# Autodesk Inventor assembly: POM_T5_07
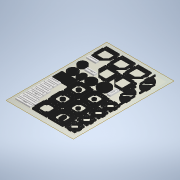
[picture p0: Inventor's stored thumbnail of the model, 180x180]
Saved by Autodesk Inventor 2020 (Build 240168000, 168)
## iProperties
Created: 2021-08-27
Part Number: POM_T5_07
Document SubType Name: Assembly
Designer: Masato
Author: Masato
## Documents named in this file (26)
- C:\Inventor\SUSTAINA-OP\Cam\POM_T5_07.iam
- C:\Inventor\SUSTAINA-OP\Cam\DisposableBoard.ipt
- C:\Inventor\SUSTAINA-OP\UpperBody\Head\Camera_root_frame_e-CAM50_CUNX.ipt
- C:\Inventor\SUSTAINA-OP\UpperBody\Arm\UpperArm_diagonal.ipt
- C:\Inventor\SUSTAINA-OP\UpperBody\Head\Camera_side_frame.ipt
- C:\Inventor\SUSTAINA-OP\SandBlastingJig\Trunk_servo_bottom_frame_SandBlastingJig.ipt
- C:\Inventor\SUSTAINA-OP\SandBlastingJig\Foot_front_frame_SandBlastingJig_back.ipt
- C:\Inventor\SUSTAINA-OP\SandBlastingJig\Foot_front_frame_SandBlastingJig_front.ipt
- C:\Inventor\SUSTAINA-OP\SandBlastingJig\Leg_joint_slider_frame_SandBlastingJig_axis_back.ipt
- C:\Inventor\SUSTAINA-OP\SandBlastingJig\Leg_joint_slider_frame_SandBlastingJig_axis_front.ipt
- C:\Inventor\SUSTAINA-OP\SandBlastingJig\Leg_joint_slider_frame_SandBlastingJig_slider_back.ipt
- C:\Inventor\SUSTAINA-OP\SandBlastingJig\Leg_joint_slider_frame_SandBlastingJig_slider_front.ipt
- C:\Inventor\SUSTAINA-OP\SandBlastingJig\Leg_joint_yaw_frame_SandBlastingJig.ipt
- C:\Inventor\SUSTAINA-OP\SandBlastingJig\Outer_support_stand_SandBlastingJig.ipt
- C:\Inventor\SUSTAINA-OP\SandBlastingJig\Shoulder_horn_frame_SandBlastingJig.ipt
- C:\Inventor\SUSTAINA-OP\SandBlastingJig\Trunk_neck_frame_AND_Trunk_shoulder_frame_SandBlastingJig.ipt
- C:\Inventor\SUSTAINA-OP\UpperBody\Arm\ForeArm_diagonal.ipt
- C:\Inventor\SUSTAINA-OP\Jig\BackLink_diagonal_Jig.ipt
- C:\Inventor\SUSTAINA-OP\Jig\Leg_joint_yaw_frame_Jig.ipt
- C:\Inventor\SUSTAINA-OP\Jig\Trunk_lower_side_frame_Jig.ipt
- C:\Inventor\SUSTAINA-OP\Jig\FrontLink_diagonal_Jig.ipt
- C:\Inventor\SUSTAINA-OP\Jig\Trunk_chest_frame_Jig_1.ipt
- C:\Inventor\SUSTAINA-OP\Jig\UpperArm_diagonal_Jig.ipt
- C:\Inventor\SUSTAINA-OP\Jig\Head_horn_frame_Jig.ipt
- C:\Inventor\SUSTAINA-OP\Jig\Shoulder_horn_frame_Jig.ipt
- C:\Inventor\SUSTAINA-OP\Jig\Foot_root_block_Jig.ipt
## Components (43 placed, 25 different names)
1. DisposableBoard:1 — メイト:2, メイト:1, フラッシュ:1, フラッシュ:2, メイト:4, メイト:5, メイト:6, メイト:7, メイト:8, メイト:9, メイト:13, メイト:14, メイト:16, メイト:17, メイト:20, メイト:22, メイト:23, メイト:25, メイト:26, メイト:27, メイト:28, 角度:1, 角度:2, 角度:3, 角度:4, メイト:29, 角度:5, メイト:30, メイト:31, メイト:32, メイト:33, メイト:34, メイト:35, フラッシュ:3, フラッシュ:4, 角度:6, 角度:7, 角度:8, 角度:9, 角度:10, 正接:11, 正接:19, メイト:36, フラッシュ:5, フラッシュ:6, メイト:38, メイト:41, フラッシュ:7, メイト:49, 角度:11, メイト:52, メイト:54, フラッシュ:9, フラッシュ:10, メイト:55, メイト:57, メイト:59, メイト:61, メイト:63, メイト:65, メイト:67, メイト:69
2. Camera_side_frame:1 — メイト:13, メイト:14, メイト:15, メイト:19
3. Camera_side_frame:4 — メイト:17, メイト:20, メイト:24, メイト:50
4. Camera_side_frame:5 — メイト:16, メイト:19, メイト:40, メイト:50, フラッシュ:8
5. Camera_side_frame:6 — メイト:22, メイト:23, メイト:24, フラッシュ:8
6. Trunk_servo_bottom_frame_SandBlastingJig:1 — メイト:30, フラッシュ:3, フラッシュ:4, 正接:12, 正接:13
7. Foot_front_frame_SandBlastingJig_back:1 — メイト:26, 角度:3, 正接:5, 正接:6
8. Foot_front_frame_SandBlastingJig_front:1 — メイト:25, 角度:2, 正接:1, 正接:2
9. Leg_joint_slider_frame_SandBlastingJig_axis_back:1 — メイト:27, 角度:4, 正接:7, 正接:8
10. Leg_joint_slider_frame_SandBlastingJig_axis_front:1 — メイト:28, 角度:1, 正接:3, 正接:4
11. Leg_joint_slider_frame_SandBlastingJig_slider_back:1 — メイト:29, 角度:5, 正接:9, 正接:10
12. Leg_joint_slider_frame_SandBlastingJig_slider_front:1 — メイト:32, 角度:7, 正接:13, 正接:14, 正接:15
13. Leg_joint_yaw_frame_SandBlastingJig:1 — メイト:33, 角度:10, 正接:19, 正接:20, 正接:21
14. Outer_support_stand_SandBlastingJig:1 — メイト:35, 角度:9, 正接:17, 正接:18, 正接:22
15. Shoulder_horn_frame_SandBlastingJig:1 — メイト:34, 角度:8, 正接:15, 正接:16, 正接:17
16. Trunk_neck_frame_AND_Trunk_shoulder_frame_SandBlastingJig:1 — メイト:31, 角度:6, 正接:11, 正接:12, 正接:14, 正接:20
17. BackLink_diagonal_Jig:1 — メイト:41, フラッシュ:7, メイト:46
18. Leg_joint_yaw_frame_Jig:1 — メイト:49, メイト:51, 角度:11, 正接:21
19. Leg_joint_yaw_frame_Jig:2 — メイト:52, メイト:53, 正接:22
20. Trunk_lower_side_frame_Jig:1 — メイト:54, フラッシュ:9, フラッシュ:10, メイト:56, フラッシュ:11
21. FrontLink_diagonal_Jig:1 — メイト:55, メイト:56, フラッシュ:11, メイト:58, フラッシュ:12
22. Trunk_chest_frame_Jig_1:1 — メイト:57, メイト:58, フラッシュ:12, メイト:60, フラッシュ:13
23. UpperArm_diagonal_Jig:1 — メイト:59, メイト:60, フラッシュ:13, メイト:62, フラッシュ:14
24. Head_horn_frame_Jig:1 — メイト:61, メイト:62, フラッシュ:14, メイト:64, フラッシュ:15
25. Shoulder_horn_frame_Jig:1 — メイト:63, メイト:64, フラッシュ:15, メイト:66, フラッシュ:16
26. BackLink_diagonal_Jig:2 — メイト:65, メイト:66, フラッシュ:16, メイト:68, フラッシュ:17
27. Leg_joint_yaw_frame_Jig:3 — メイト:67, メイト:68, フラッシュ:17, メイト:70, フラッシュ:18
28. Foot_root_block_Jig:1 — メイト:69, メイト:70, フラッシュ:18
29. UpperArm_diagonal:1 — メイト:7, メイト:8, メイト:9
30. UpperArm_diagonal:2
31. UpperArm_diagonal:3
32. UpperArm_diagonal:4 — メイト:15
33. ForeArm_diagonal:1 — メイト:36, フラッシュ:5, フラッシュ:6, メイト:46
34. ForeArm_diagonal:2
35. ForeArm_diagonal:3 — メイト:39
36. ForeArm_diagonal:4 — メイト:38, メイト:39, メイト:40, メイト:53
37. ForeArm_diagonal:5 — メイト:51
38. Camera_root_frame_e-CAM50_CUNX:1 — メイト:4, メイト:5, メイト:6
39. Camera_root_frame_e-CAM50_CUNX:2 — 正接:9, 正接:10
40. Camera_root_frame_e-CAM50_CUNX:3 — 正接:1, 正接:2
41. Camera_root_frame_e-CAM50_CUNX:4 — 正接:3, 正接:4
42. Camera_root_frame_e-CAM50_CUNX:5 — 正接:5, 正接:6, 正接:16
43. Camera_root_frame_e-CAM50_CUNX:6 — 正接:7, 正接:8, 正接:18
## Component patterns: (4 elements, first: UpperArm_diagonal:1), (3 elements), (3 elements, first: ForeArm_diagonal:1), (2 elements, first: ForeArm_diagonal:4), (2 elements, first: Camera_root_frame_e-CAM50_CUNX:1), コンポーネント パターン 7:2 (2 elements), コンポーネント パターン 7:3 (2 elements)
## Relationships (108: Mate 57, Tangent 22, Flush 18, Angle 11)
- メイト:2 [Mate]: DisposableBoard:1
- メイト:1 [Mate]: DisposableBoard:1
- フラッシュ:1 [Flush]: DisposableBoard:1
- フラッシュ:2 [Flush]: DisposableBoard:1
- メイト:4 [Mate]: DisposableBoard:1 ↔ Camera_root_frame_e-CAM50_CUNX:1
- メイト:5 [Mate] (2 mm): DisposableBoard:1 ↔ Camera_root_frame_e-CAM50_CUNX:1
- メイト:6 [Mate] (56.2 mm): DisposableBoard:1 ↔ Camera_root_frame_e-CAM50_CUNX:1
- メイト:7 [Mate]: DisposableBoard:1 ↔ UpperArm_diagonal:1
- メイト:8 [Mate] (2 mm): DisposableBoard:1 ↔ UpperArm_diagonal:1
- メイト:9 [Mate] (2 mm): DisposableBoard:1 ↔ UpperArm_diagonal:1
- メイト:13 [Mate]: DisposableBoard:1 ↔ Camera_side_frame:1
- メイト:14 [Mate] (5 mm): DisposableBoard:1 ↔ Camera_side_frame:1
- メイト:15 [Mate] (2.5 mm): Camera_side_frame:1 ↔ UpperArm_diagonal:4
- メイト:16 [Mate]: DisposableBoard:1 ↔ Camera_side_frame:5
- メイト:17 [Mate]: DisposableBoard:1 ↔ Camera_side_frame:4
- メイト:19 [Mate] (10 mm): Camera_side_frame:1 ↔ Camera_side_frame:5
- メイト:20 [Mate] (5 mm): DisposableBoard:1 ↔ Camera_side_frame:4
- メイト:22 [Mate]: DisposableBoard:1 ↔ Camera_side_frame:6
- メイト:23 [Mate] (2 mm): DisposableBoard:1 ↔ Camera_side_frame:6
- メイト:24 [Mate] (9 mm): Camera_side_frame:4 ↔ Camera_side_frame:6
- メイト:25 [Mate]: DisposableBoard:1 ↔ Foot_front_frame_SandBlastingJig_front:1
- メイト:26 [Mate]: DisposableBoard:1 ↔ Foot_front_frame_SandBlastingJig_back:1
- メイト:27 [Mate]: DisposableBoard:1 ↔ Leg_joint_slider_frame_SandBlastingJig_axis_back:1
- メイト:28 [Mate]: DisposableBoard:1 ↔ Leg_joint_slider_frame_SandBlastingJig_axis_front:1
- 角度:1 [Angle] (0 deg): DisposableBoard:1 ↔ Leg_joint_slider_frame_SandBlastingJig_axis_front:1
- 角度:2 [Angle] (0 deg): DisposableBoard:1 ↔ Foot_front_frame_SandBlastingJig_front:1
- 角度:3 [Angle] (0 deg): DisposableBoard:1 ↔ Foot_front_frame_SandBlastingJig_back:1
- 角度:4 [Angle] (0 deg): DisposableBoard:1 ↔ Leg_joint_slider_frame_SandBlastingJig_axis_back:1
- 正接:1 [Tangent] (7.5 mm): Foot_front_frame_SandBlastingJig_front:1 ↔ Camera_root_frame_e-CAM50_CUNX:3
- 正接:2 [Tangent] (7.5 mm): Foot_front_frame_SandBlastingJig_front:1 ↔ Camera_root_frame_e-CAM50_CUNX:3
- 正接:3 [Tangent] (7.5 mm): Leg_joint_slider_frame_SandBlastingJig_axis_front:1 ↔ Camera_root_frame_e-CAM50_CUNX:4
- 正接:4 [Tangent] (7.5 mm): Leg_joint_slider_frame_SandBlastingJig_axis_front:1 ↔ Camera_root_frame_e-CAM50_CUNX:4
- 正接:5 [Tangent] (7.5 mm): Foot_front_frame_SandBlastingJig_back:1 ↔ Camera_root_frame_e-CAM50_CUNX:5
- 正接:6 [Tangent] (7.5 mm): Foot_front_frame_SandBlastingJig_back:1 ↔ Camera_root_frame_e-CAM50_CUNX:5
- 正接:7 [Tangent] (7.5 mm): Leg_joint_slider_frame_SandBlastingJig_axis_back:1 ↔ Camera_root_frame_e-CAM50_CUNX:6
- 正接:8 [Tangent] (7.5 mm): Leg_joint_slider_frame_SandBlastingJig_axis_back:1 ↔ Camera_root_frame_e-CAM50_CUNX:6
- メイト:29 [Mate]: DisposableBoard:1 ↔ Leg_joint_slider_frame_SandBlastingJig_slider_back:1
- 角度:5 [Angle] (0 deg): DisposableBoard:1 ↔ Leg_joint_slider_frame_SandBlastingJig_slider_back:1
- 正接:9 [Tangent] (2.5 mm): Leg_joint_slider_frame_SandBlastingJig_slider_back:1 ↔ Camera_root_frame_e-CAM50_CUNX:2
- 正接:10 [Tangent] (5.5 mm): Leg_joint_slider_frame_SandBlastingJig_slider_back:1 ↔ Camera_root_frame_e-CAM50_CUNX:2
- メイト:30 [Mate]: DisposableBoard:1 ↔ Trunk_servo_bottom_frame_SandBlastingJig:1
- メイト:31 [Mate]: DisposableBoard:1 ↔ Trunk_neck_frame_AND_Trunk_shoulder_frame_SandBlastingJig:1
- メイト:32 [Mate]: DisposableBoard:1 ↔ Leg_joint_slider_frame_SandBlastingJig_slider_front:1
- メイト:33 [Mate]: DisposableBoard:1 ↔ Leg_joint_yaw_frame_SandBlastingJig:1
- メイト:34 [Mate]: DisposableBoard:1 ↔ Shoulder_horn_frame_SandBlastingJig:1
- メイト:35 [Mate]: DisposableBoard:1 ↔ Outer_support_stand_SandBlastingJig:1
- フラッシュ:3 [Flush] (124.25 mm): DisposableBoard:1 ↔ Trunk_servo_bottom_frame_SandBlastingJig:1
- フラッシュ:4 [Flush] (2.5 mm): DisposableBoard:1 ↔ Trunk_servo_bottom_frame_SandBlastingJig:1
- 角度:6 [Angle] (0 deg): DisposableBoard:1 ↔ Trunk_neck_frame_AND_Trunk_shoulder_frame_SandBlastingJig:1
- 角度:7 [Angle] (90 deg): DisposableBoard:1 ↔ Leg_joint_slider_frame_SandBlastingJig_slider_front:1
- 角度:8 [Angle] (0 deg): DisposableBoard:1 ↔ Shoulder_horn_frame_SandBlastingJig:1
- 角度:9 [Angle] (0 deg): DisposableBoard:1 ↔ Outer_support_stand_SandBlastingJig:1
- 角度:10 [Angle] (0 deg): DisposableBoard:1 ↔ Leg_joint_yaw_frame_SandBlastingJig:1
- 正接:11 [Tangent] (2.5 mm): DisposableBoard:1 ↔ Trunk_neck_frame_AND_Trunk_shoulder_frame_SandBlastingJig:1
- 正接:12 [Tangent] (2.5 mm): Trunk_servo_bottom_frame_SandBlastingJig:1 ↔ Trunk_neck_frame_AND_Trunk_shoulder_frame_SandBlastingJig:1
- 正接:13 [Tangent] (2.5 mm): Trunk_servo_bottom_frame_SandBlastingJig:1 ↔ Leg_joint_slider_frame_SandBlastingJig_slider_front:1
- 正接:14 [Tangent] (2.5 mm): Leg_joint_slider_frame_SandBlastingJig_slider_front:1 ↔ Trunk_neck_frame_AND_Trunk_shoulder_frame_SandBlastingJig:1
- 正接:15 [Tangent] (2.5 mm): Leg_joint_slider_frame_SandBlastingJig_slider_front:1 ↔ Shoulder_horn_frame_SandBlastingJig:1
- 正接:16 [Tangent] (2.5 mm): Shoulder_horn_frame_SandBlastingJig:1 ↔ Camera_root_frame_e-CAM50_CUNX:5
- 正接:17 [Tangent] (2.5 mm): Outer_support_stand_SandBlastingJig:1 ↔ Shoulder_horn_frame_SandBlastingJig:1
- 正接:18 [Tangent] (2.5 mm): Outer_support_stand_SandBlastingJig:1 ↔ Camera_root_frame_e-CAM50_CUNX:6
- 正接:19 [Tangent] (2.5 mm): DisposableBoard:1 ↔ Leg_joint_yaw_frame_SandBlastingJig:1
- 正接:20 [Tangent] (2.5 mm): Leg_joint_yaw_frame_SandBlastingJig:1 ↔ Trunk_neck_frame_AND_Trunk_shoulder_frame_SandBlastingJig:1
- メイト:36 [Mate]: DisposableBoard:1 ↔ ForeArm_diagonal:1
- フラッシュ:5 [Flush] (1.5 mm): DisposableBoard:1 ↔ ForeArm_diagonal:1
- フラッシュ:6 [Flush] (3.5 mm): DisposableBoard:1 ↔ ForeArm_diagonal:1
- メイト:38 [Mate]: DisposableBoard:1 ↔ ForeArm_diagonal:4
- メイト:39 [Mate] (2.5 mm): ForeArm_diagonal:3 ↔ ForeArm_diagonal:4
- メイト:40 [Mate] (2.5 mm): Camera_side_frame:5 ↔ ForeArm_diagonal:4
- メイト:41 [Mate]: DisposableBoard:1 ↔ BackLink_diagonal_Jig:1
- フラッシュ:7 [Flush] (2.5 mm): DisposableBoard:1 ↔ BackLink_diagonal_Jig:1
- メイト:46 [Mate] (2.5 mm): BackLink_diagonal_Jig:1 ↔ ForeArm_diagonal:1
- メイト:49 [Mate]: DisposableBoard:1 ↔ Leg_joint_yaw_frame_Jig:1
- メイト:50 [Mate] (22 mm): Camera_side_frame:4 ↔ Camera_side_frame:5
- フラッシュ:8 [Flush]: Camera_side_frame:5 ↔ Camera_side_frame:6
- メイト:51 [Mate] (2.5 mm): Leg_joint_yaw_frame_Jig:1 ↔ ForeArm_diagonal:5
- 角度:11 [Angle] (0 deg): DisposableBoard:1 ↔ Leg_joint_yaw_frame_Jig:1
- 正接:21 [Tangent] (2.5 mm): Leg_joint_yaw_frame_SandBlastingJig:1 ↔ Leg_joint_yaw_frame_Jig:1
- メイト:52 [Mate]: DisposableBoard:1 ↔ Leg_joint_yaw_frame_Jig:2
- メイト:53 [Mate] (2.5 mm): Leg_joint_yaw_frame_Jig:2 ↔ ForeArm_diagonal:4
- 正接:22 [Tangent] (2.5 mm): Outer_support_stand_SandBlastingJig:1 ↔ Leg_joint_yaw_frame_Jig:2
- メイト:54 [Mate]: DisposableBoard:1 ↔ Trunk_lower_side_frame_Jig:1
- フラッシュ:9 [Flush] (2.5 mm): DisposableBoard:1 ↔ Trunk_lower_side_frame_Jig:1
- フラッシュ:10 [Flush] (2.5 mm): DisposableBoard:1 ↔ Trunk_lower_side_frame_Jig:1
- メイト:55 [Mate]: DisposableBoard:1 ↔ FrontLink_diagonal_Jig:1
- メイト:56 [Mate] (2.5 mm): Trunk_lower_side_frame_Jig:1 ↔ FrontLink_diagonal_Jig:1
- フラッシュ:11 [Flush]: Trunk_lower_side_frame_Jig:1 ↔ FrontLink_diagonal_Jig:1
- メイト:57 [Mate]: DisposableBoard:1 ↔ Trunk_chest_frame_Jig_1:1
- メイト:58 [Mate] (2.5 mm): FrontLink_diagonal_Jig:1 ↔ Trunk_chest_frame_Jig_1:1
- フラッシュ:12 [Flush]: FrontLink_diagonal_Jig:1 ↔ Trunk_chest_frame_Jig_1:1
- メイト:59 [Mate]: DisposableBoard:1 ↔ UpperArm_diagonal_Jig:1
- メイト:60 [Mate] (2.5 mm): Trunk_chest_frame_Jig_1:1 ↔ UpperArm_diagonal_Jig:1
- フラッシュ:13 [Flush]: Trunk_chest_frame_Jig_1:1 ↔ UpperArm_diagonal_Jig:1
- メイト:61 [Mate]: DisposableBoard:1 ↔ Head_horn_frame_Jig:1
- メイト:62 [Mate] (2.5 mm): UpperArm_diagonal_Jig:1 ↔ Head_horn_frame_Jig:1
- フラッシュ:14 [Flush]: UpperArm_diagonal_Jig:1 ↔ Head_horn_frame_Jig:1
- メイト:63 [Mate]: DisposableBoard:1 ↔ Shoulder_horn_frame_Jig:1
- メイト:64 [Mate] (2.5 mm): Head_horn_frame_Jig:1 ↔ Shoulder_horn_frame_Jig:1
- フラッシュ:15 [Flush]: Head_horn_frame_Jig:1 ↔ Shoulder_horn_frame_Jig:1
- メイト:65 [Mate]: DisposableBoard:1 ↔ BackLink_diagonal_Jig:2
- メイト:66 [Mate] (2.5 mm): Shoulder_horn_frame_Jig:1 ↔ BackLink_diagonal_Jig:2
- フラッシュ:16 [Flush]: Shoulder_horn_frame_Jig:1 ↔ BackLink_diagonal_Jig:2
- メイト:67 [Mate]: DisposableBoard:1 ↔ Leg_joint_yaw_frame_Jig:3
- メイト:68 [Mate] (2.5 mm): BackLink_diagonal_Jig:2 ↔ Leg_joint_yaw_frame_Jig:3
- フラッシュ:17 [Flush]: BackLink_diagonal_Jig:2 ↔ Leg_joint_yaw_frame_Jig:3
- メイト:69 [Mate]: DisposableBoard:1 ↔ Foot_root_block_Jig:1
- メイト:70 [Mate] (2.5 mm): Leg_joint_yaw_frame_Jig:3 ↔ Foot_root_block_Jig:1
- フラッシュ:18 [Flush]: Leg_joint_yaw_frame_Jig:3 ↔ Foot_root_block_Jig:1
